# Autodesk Inventor assembly: tower_MIR
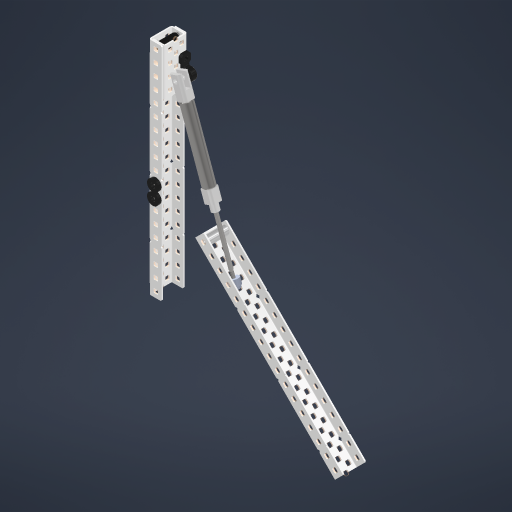
[picture p0: Inventor's stored thumbnail of the model, 512x512]
Saved by Autodesk Inventor 2024 (Build 280153000, 153)
## iProperties
Created: 2024-01-16
Part Number: tower_MIR
Document SubType Name: Assembly
Designer: Averey Ku
Author: avere
## Documents named in this file (16)
- C:\Users\avere\Documents\rbp_cad\zoomba_v0.3\tower\mirrored_parts\tower_MIR.iam
- C:\Users\avere\Documents\rbp_cad\zoomba_v0.3\tower\mirrored_parts\Alu C 1x2x1x19_MIR.ipt
- C:\Users\avere\Documents\rbp_cad\zoomba_v0.3\tower\mirrored_parts\Alu C 1x2x1x4_MIR.ipt
- C:\Users\avere\Documents\rbp_cad\VEX-CAD-Inventor-1.41\Motion\Spacers\Spacer Nylon .500 OD\NSpacer Black .500 OD x .125.ipt
- C:\Users\avere\Documents\rbp_cad\zoomba_v0.3\tower\mirrored_parts\LS Pillow Bearing Block_MIR.ipt
- C:\Users\avere\Documents\rbp_cad\zoomba_v0.3\tower\mirrored_parts\Double Acting Piston_MIR.iam
- C:\Users\avere\Documents\rbp_cad\zoomba_v0.3\tower\mirrored_parts\Alu C 1x2x1x17_MIR.ipt
- C:\Users\avere\Documents\rbp_cad\zoomba_v0.3\tower\mirrored_parts\Shaft Collar No Screw_MIR.ipt
- C:\Users\avere\Documents\rbp_cad\zoomba_v0.3\tower\mirrored_parts\Piston Nut_MIR.ipt
- C:\Users\avere\Documents\rbp_cad\zoomba_v0.3\tower\mirrored_parts\.375 OD Aluminum Spacer 0.875_MIR.ipt
- C:\Users\avere\Documents\rbp_cad\VEX-CAD-Inventor-1.41\Motion\Spacers\Spacer Nylon .500 OD.ipt
- C:\Users\avere\Documents\rbp_cad\VEX-CAD-Inventor-1.41\Motion\Spacers\Spacer Nylon .375 OD\NSpacer .375 OD x .500.ipt
- C:\Users\avere\Documents\rbp_cad\VEX-CAD-Inventor-1.41\Motion\Spacers\Spacer Nylon .375 OD.ipt
- C:\Users\avere\Documents\rbp_cad\VEX-CAD-Inventor-1.41\Motion\Spacers\Spacer Nylon .375 OD\NSpacer .375 OD x .250.ipt
- C:\Users\avere\Documents\rbp_cad\VEX-CAD-Inventor-1.41\Motion\Spacers\Washer Steel\SWasher .375 OD x .062500.ipt
- C:\Users\avere\Documents\rbp_cad\VEX-CAD-Inventor-1.41\Motion\Spacers\Washer Steel.ipt
## Components (13 placed, 12 different names)
1. Alu C 1x2x1x19_MIR:1 — Mate:1, Insert:1, Insert:4, Insert:3, Angle:1, Insert:14
2. Alu C 1x2x1x4_MIR:1 — Mate:1, Insert:1, Mate:2, Insert:5
3. NSpacer Black .500 OD x .125:1 — Insert:4
4. NSpacer Black .500 OD x .125:2 — Insert:3
5. LS Pillow Bearing Block_MIR:1 — Mate:2, Insert:5, Insert:9
6. Double Acting Piston_MIR:1 [sub-assembly] — Insert:9, Insert:11
7. Alu C 1x2x1x17_MIR:1 — Angle:1, Mate:3, Insert:12
8. Shaft Collar No Screw_MIR:1 — Mate:3, Insert:10
9. Piston Nut_MIR:1 — Insert:11, Insert:10
10. .375 OD Aluminum Spacer 0.875_MIR:1 — Insert:12
11. NSpacer .375 OD x .500:1 — Insert:12
12. NSpacer .375 OD x .250:2 — Insert:12, Insert:13
13. SWasher .375 OD x .062500:1 — Insert:13, Insert:14
## Relationships (15: Insert 11, Mate 3, Angle 1)
- Mate:1: Alu C 1x2x1x19_MIR:1 ↔ Alu C 1x2x1x4_MIR:1
- Insert:1: Alu C 1x2x1x19_MIR:1 ↔ Alu C 1x2x1x4_MIR:1
- Insert:4: Alu C 1x2x1x19_MIR:1 ↔ NSpacer Black .500 OD x .125:1
- Insert:3: Alu C 1x2x1x19_MIR:1 ↔ NSpacer Black .500 OD x .125:2
- Mate:2: Alu C 1x2x1x4_MIR:1 ↔ LS Pillow Bearing Block_MIR:1
- Insert:5 (1.5875 mm): Alu C 1x2x1x4_MIR:1 ↔ LS Pillow Bearing Block_MIR:1
- Insert:9: LS Pillow Bearing Block_MIR:1 ↔ Double Acting Piston_MIR:1
- Angle:1 (0 deg): Alu C 1x2x1x19_MIR:1 ↔ Alu C 1x2x1x17_MIR:1
- Mate:3: Alu C 1x2x1x17_MIR:1 ↔ Shaft Collar No Screw_MIR:1
- Insert:11: Double Acting Piston_MIR:1 ↔ Piston Nut_MIR:1
- Insert:10: Shaft Collar No Screw_MIR:1 ↔ Piston Nut_MIR:1
- Insert:12: Alu C 1x2x1x17_MIR:1 ↔ .375 OD Aluminum Spacer 0.875_MIR:1
- Insert:12: NSpacer .375 OD x .500:1 ↔ NSpacer .375 OD x .250:2
- Insert:13: NSpacer .375 OD x .250:2 ↔ SWasher .375 OD x .062500:1
- Insert:14: Alu C 1x2x1x19_MIR:1 ↔ SWasher .375 OD x .062500:1
